# Autodesk Inventor assembly: Rail_assy
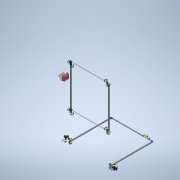
[picture p0: Inventor's stored thumbnail of the model, 180x180]
Saved by Autodesk Inventor 2021 (Build 250183000, 183)
## iProperties
Created: 2021-02-01
Part Number: Rail_assy
Document SubType Name: Assembly
Designer: Jorian Brusind
Author: Jorian Brusind
## Documents named in this file (13)
- C:\Users\Jorian Brusind\Documents\GitHub\PersonalProjects\HyperRail\Inventor Files\Rail_assy.iam
- C:\Users\Jorian Brusind\Documents\GitHub\PersonalProjects\HyperRail\Inventor Files\Rail_Assembly.iam
- C:\Users\Jorian Brusind\Documents\GitHub\PersonalProjects\HyperRail\Inventor Files\YAxis_Carriage.iam
- C:\Users\Jorian Brusind\Documents\GitHub\PersonalProjects\HyperRail\Inventor Files\Small_belt_5mm_1mm.ipt
- C:\Users\Jorian Brusind\Documents\GitHub\PersonalProjects\HyperRail\Inventor Files\90deg_4040Bracket.ipt
- C:\Users\Jorian Brusind\Documents\GitHub\PersonalProjects\Inventor Projects\Useful models\8020_Sets\IPT_20_Series\Extra_20_Series\8020_14057m\14057_m.ipt
- C:\Users\Jorian Brusind\Documents\GitHub\PersonalProjects\HyperRail\Inventor Files\Small_Belt_Clamp.ipt
- C:\Users\Jorian Brusind\Documents\GitHub\PersonalProjects\HyperRail\Inventor Files\Ebox_assy.iam
- C:\Users\Jorian Brusind\Documents\GitHub\PersonalProjects\HyperRail\Inventor Files\RightAngle_Bracket.ipt
- C:\Users\Jorian Brusind\Documents\GitHub\PersonalProjects\Inventor Projects\Useful models\8020_Sets\IPT_40_Series\Extra_40_Series\90deg_4040.ipt
- C:\Users\Jorian Brusind\Documents\GitHub\PersonalProjects\HyperRail\PCB Files\Integrated Stepper Motor Driver\ExportSTEP\Main.iam
- C:\Users\Jorian Brusind\Documents\GitHub\PersonalProjects\Inventor Projects\Useful models\8020_Sets\IPT_20_Series\IPT_20_Series\20-2040_2m.ipt
- C:\Users\Jorian Brusind\Documents\GitHub\PersonalProjects\Inventor Projects\Useful models\8020_Sets\IPT_20_Series\IPT_20_Series\20-2020_variable.ipt
## Components (25 placed, 12 different names)
1. Rail_Assembly:1 [sub-assembly] — Mate:48, Flush:38, Flush:39, Flush:40, Flush:41, Flush:46, Flush:47, Mate:52, Mate:55, Flush:54, Mate:57, Flush:56, Mate:58, Flush:57, Mate:64, Mate:66, Flush:62, Mate:70
2. YAxis_Carriage:1 [sub-assembly] — Mate:11, Mate:15, Mate:46, Flush:34, Flush:35, Flush:65, Mate:72
3. Rail_Assembly:2 [sub-assembly] — Mate:47, Flush:36, Flush:37, Flush:40, Flush:41, Mate:53, Flush:48, Flush:49, Flush:50, Mate:54, Flush:51, Flush:52, Flush:53, Mate:59, Mate:61, Flush:60, Mate:71, Mate:75, Flush:68, Mate:77, Flush:69, Mate:78, Flush:71
4. Small_belt_5mm_1mm:1 — Mate:11, Flush:66, Flush:67
5. Small_belt_5mm_1mm:2 — Mate:15, Mate:73, Mate:74, Flush:66, Flush:67
6. 90deg_4040Bracket:2 — Mate:77, Flush:69, Flush:70
7. 14057_m:1
8. 90deg_4040Bracket:3 — Mate:57, Flush:55, Flush:56
9. 90deg_4040Bracket:4 — Mate:58, Flush:57, Flush:58
10. Small_Belt_Clamp:1
11. Small_Belt_Clamp:2 — Mate:67, Flush:63, Flush:64
12. Ebox_assy:1 [sub-assembly]
13. RightAngle_Bracket:1 — Mate:61, Mate:62, Flush:60
14. RightAngle_Bracket:2 — Mate:59, Mate:60, Flush:59
15. RightAngle_Bracket:3 — Mate:63, Mate:64, Flush:61
16. RightAngle_Bracket:4 — Mate:65, Mate:66, Flush:62
17. 90deg_4040:1 — Mate:75, Flush:68, Mate:76
18. 90deg_4040:2 — Mate:55, Mate:56, Flush:54
19. Main:1 [sub-assembly] — Mate:46, Flush:34, Flush:35
20. Main:2 [sub-assembly] — Mate:47, Flush:36, Flush:37
21. Main:3 [sub-assembly] — Mate:48, Flush:38, Flush:39
22. 20-2040_2m:1 — Flush:46, Flush:47, Mate:52, Flush:52, Flush:53, Mate:56, Flush:55, Flush:58, Mate:67, Flush:63, Flush:64, Flush:65, Mate:72, Mate:73, Mate:74, Mate:76, Flush:70, Flush:72
23. 20-2020_variable:1 — Flush:50, Mate:54, Flush:51, Mate:60, Flush:59, Mate:65, Mate:69
24. 20-2020_variable:2 — Mate:53, Flush:48, Flush:49, Mate:62, Mate:63, Flush:61
25. 90deg_4040Bracket:5 — Mate:78, Flush:71, Flush:72
## Relationships (66: Flush 35, Mate 31)
- Mate:11: YAxis_Carriage:1 ↔ Small_belt_5mm_1mm:1
- Mate:15: YAxis_Carriage:1 ↔ Small_belt_5mm_1mm:2
- Mate:46: YAxis_Carriage:1 ↔ Main:1
- Flush:34: YAxis_Carriage:1 ↔ Main:1
- Flush:35: YAxis_Carriage:1 ↔ Main:1
- Mate:47: Rail_Assembly:2 ↔ Main:2
- Flush:36 (7.5 mm): Rail_Assembly:2 ↔ Main:2
- Flush:37 (7.5 mm): Rail_Assembly:2 ↔ Main:2
- Mate:48: Rail_Assembly:1 ↔ Main:3
- Flush:38 (7.5 mm): Rail_Assembly:1 ↔ Main:3
- Flush:39 (7.5 mm): Rail_Assembly:1 ↔ Main:3
- Flush:40: Rail_Assembly:1 ↔ Rail_Assembly:2
- Flush:41: Rail_Assembly:1 ↔ Rail_Assembly:2
- Flush:46: Rail_Assembly:1 ↔ 20-2040_2m:1
- Flush:47: Rail_Assembly:1 ↔ 20-2040_2m:1
- Mate:52: Rail_Assembly:1 ↔ 20-2040_2m:1
- Mate:53: Rail_Assembly:2 ↔ 20-2020_variable:2
- Flush:48: Rail_Assembly:2 ↔ 20-2020_variable:2
- Flush:49: Rail_Assembly:2 ↔ 20-2020_variable:2
- Flush:50: Rail_Assembly:2 ↔ 20-2020_variable:1
- Mate:54: Rail_Assembly:2 ↔ 20-2020_variable:1
- Flush:51: Rail_Assembly:2 ↔ 20-2020_variable:1
- Flush:52: Rail_Assembly:2 ↔ 20-2040_2m:1
- Flush:53: Rail_Assembly:2 ↔ 20-2040_2m:1
- Mate:55: Rail_Assembly:1 ↔ 90deg_4040:2
- Mate:56: 90deg_4040:2 ↔ 20-2040_2m:1
- Flush:54: Rail_Assembly:1 ↔ 90deg_4040:2
- Mate:57: Rail_Assembly:1 ↔ 90deg_4040Bracket:3
- Flush:55: 90deg_4040Bracket:3 ↔ 20-2040_2m:1
- Flush:56: Rail_Assembly:1 ↔ 90deg_4040Bracket:3
- Mate:58: Rail_Assembly:1 ↔ 90deg_4040Bracket:4
- Flush:57: Rail_Assembly:1 ↔ 90deg_4040Bracket:4
- Flush:58: 90deg_4040Bracket:4 ↔ 20-2040_2m:1
- Mate:59: Rail_Assembly:2 ↔ RightAngle_Bracket:2
- Mate:60: RightAngle_Bracket:2 ↔ 20-2020_variable:1
- Flush:59: RightAngle_Bracket:2 ↔ 20-2020_variable:1
- Mate:61: Rail_Assembly:2 ↔ RightAngle_Bracket:1
- Mate:62: RightAngle_Bracket:1 ↔ 20-2020_variable:2
- Flush:60: Rail_Assembly:2 ↔ RightAngle_Bracket:1
- Mate:63: RightAngle_Bracket:3 ↔ 20-2020_variable:2
- Mate:64: Rail_Assembly:1 ↔ RightAngle_Bracket:3
- Flush:61: RightAngle_Bracket:3 ↔ 20-2020_variable:2
- Mate:65: RightAngle_Bracket:4 ↔ 20-2020_variable:1
- Mate:66: Rail_Assembly:1 ↔ RightAngle_Bracket:4
- Flush:62: Rail_Assembly:1 ↔ RightAngle_Bracket:4
- Mate:67: Small_Belt_Clamp:2 ↔ 20-2040_2m:1
- Flush:63: Small_Belt_Clamp:2 ↔ 20-2040_2m:1
- Flush:64: Small_Belt_Clamp:2 ↔ 20-2040_2m:1
- Flush:65: YAxis_Carriage:1 ↔ 20-2040_2m:1
- Mate:69: 20-2020_variable:1
- Mate:70: Rail_Assembly:1
- Mate:71: Rail_Assembly:2
- Mate:72 (1 mm): YAxis_Carriage:1 ↔ 20-2040_2m:1
- Mate:73: Small_belt_5mm_1mm:2 ↔ 20-2040_2m:1
- Mate:74: Small_belt_5mm_1mm:2 ↔ 20-2040_2m:1
- Flush:66: Small_belt_5mm_1mm:1 ↔ Small_belt_5mm_1mm:2
- Flush:67: Small_belt_5mm_1mm:1 ↔ Small_belt_5mm_1mm:2
- Mate:75: Rail_Assembly:2 ↔ 90deg_4040:1
- Flush:68: Rail_Assembly:2 ↔ 90deg_4040:1
- Mate:76: 90deg_4040:1 ↔ 20-2040_2m:1
- Mate:77: Rail_Assembly:2 ↔ 90deg_4040Bracket:2
- Flush:69: Rail_Assembly:2 ↔ 90deg_4040Bracket:2
- Flush:70: 90deg_4040Bracket:2 ↔ 20-2040_2m:1
- Mate:78: Rail_Assembly:2 ↔ 90deg_4040Bracket:5
- Flush:71: Rail_Assembly:2 ↔ 90deg_4040Bracket:5
- Flush:72: 20-2040_2m:1 ↔ 90deg_4040Bracket:5
